# Autodesk Inventor assembly: Сборка1
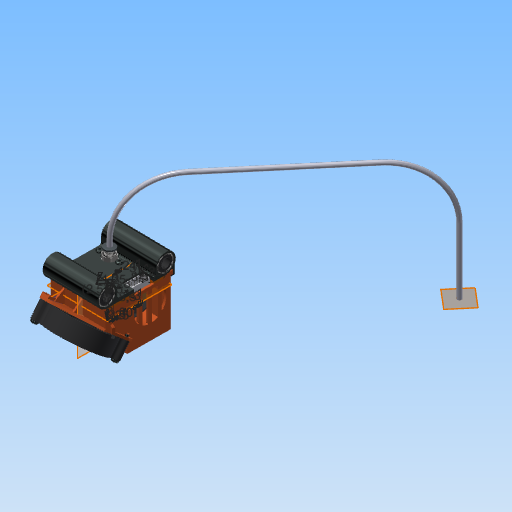
[picture p0: Inventor's stored thumbnail of the model, 512x512]
Saved by Autodesk Inventor 2017 (Build 210142000, 142)
## iProperties
Part Number: Сборка1
Material: Типовые
Document SubType Name: Assembly
Designer: Max
Author: Max
## Documents named in this file (20)
- C:\Users\Max\Desktop\Flying Bear Ghost 5\hotend assembly.iam
- C:\Users\Max\Desktop\Flying Bear Ghost 5\screw m3.ipt
- C:\Users\Max\Desktop\Flying Bear Ghost 5\linear bearing 8x15x24.ipt
- C:\Users\Max\Desktop\Flying Bear Ghost 5\hotend carriage.ipt
- C:\Users\Max\Desktop\Flying Bear Ghost 5\casing 1.ipt
- C:\Users\Max\Desktop\Flying Bear Ghost 5\casing2.ipt
- C:\Users\Max\Desktop\Flying Bear Ghost 5\hotend board.ipt
- C:\Users\Max\Desktop\Flying Bear Ghost 5\radiator Е3DV6.ipt
- C:\Users\Max\Desktop\Flying Bear Ghost 5\thermal barrier.ipt
- C:\Users\Max\Desktop\Flying Bear Ghost 5\fitting 1.ipt
- C:\Users\Max\Desktop\Flying Bear Ghost 5\heating block.ipt
- C:\Users\Max\Desktop\Flying Bear Ghost 5\nozzle 0.4 nozzle.ipt
- C:\Users\Max\Desktop\Flying Bear Ghost 5\thermal sensor.ipt
- C:\Users\Max\Desktop\Flying Bear Ghost 5\thermal sensor1.ipt
- C:\Users\Max\Desktop\Flying Bear Ghost 5\block cover.ipt
- C:\Users\Max\Desktop\Flying Bear Ghost 5\5015 snail blower fan.ipt
- C:\Users\Max\Desktop\Flying Bear Ghost 5\screw m3 long.ipt
- C:\Users\Max\Desktop\Flying Bear Ghost 5\3010-2.ipt
- C:\Users\Max\Desktop\Flying Bear Ghost 5\3010.ipt
- C:\Users\Max\Desktop\Flying Bear Ghost 5\teflon.ipt
## Components (27 placed, 19 different names)
1. hotend carriage:1 — Совмещение:276, Совмещение:277, Совмещение:278, Совмещение:279, Заподлицо:110, Заподлицо:111, Заподлицо:112, Заподлицо:113, Совмещение:282, Совмещение:283, Совмещение:285, Совмещение:287, Совмещение:288, Совмещение:290, Совмещение:291, Совмещение:292, Совмещение:298, Совмещение:299, Совмещение:300, Совмещение:301, Совмещение:317, Совмещение:318, Совмещение:319
2. linear bearing 8x15x24:5 — Совмещение:277, Заподлицо:111
3. linear bearing 8x15x24:6 — Совмещение:278, Заподлицо:110
4. linear bearing 8x15x24:7 — Совмещение:276, Заподлицо:112
5. linear bearing 8x15x24:8 — Совмещение:279, Заподлицо:113
6. casing 1:1 — Совмещение:282, Совмещение:283, Заподлицо:114, Совмещение:284, Совмещение:285, Совмещение:286, Совмещение:289, Совмещение:322
7. casing2:1 — Заподлицо:114, Совмещение:284, Совмещение:286, Угол:7, Совмещение:311, Угол:8, Совмещение:312, Совмещение:313, Совмещение:321, Угол:9
8. hotend board:1 — Совмещение:287, Совмещение:288, Совмещение:289
9. radiator Е3DV6:1 — Совмещение:290, Совмещение:291, Совмещение:292, Совмещение:293, Совмещение:294, Совмещение:297, Совмещение:436
10. thermal barrier:1 — Совмещение:293, Совмещение:294, Совмещение:302, Совмещение:304
11. fitting 1:1 — Совмещение:297, Совмещение:436, Совмещение:437
12. screw m3:45 — Совмещение:298, Совмещение:300
13. screw m3:46 — Совмещение:299, Совмещение:301
14. heating block:1 — Совмещение:302, Совмещение:303, Угол:7, Совмещение:305, Совмещение:306, Заподлицо:116, Совмещение:307, Заподлицо:117, Совмещение:309, Совмещение:310
15. nozzle 0.4 nozzle:1 — Совмещение:303, Совмещение:304, Совмещение:305, Совмещение:308
16. thermal sensor:1 — Совмещение:306, Заподлицо:116
17. thermal sensor1:1 — Совмещение:307, Заподлицо:117
18. block cover:1 — Совмещение:308, Совмещение:309, Совмещение:310
19. 5015 snail blower fan:1 — Совмещение:311, Угол:8, Совмещение:312, Совмещение:313, Совмещение:314, Совмещение:315, Совмещение:316
20. screw m3 long:1 — Совмещение:314, Совмещение:315, Заподлицо:118
21. screw m3 long:2 — Совмещение:316, Заподлицо:118
22. screw m3 long:3 — Совмещение:318, Заподлицо:119
23. screw m3 long:4 — Совмещение:317, Заподлицо:119, Совмещение:319
24. 3010-2:1 — Совмещение:320, Заподлицо:120, Совмещение:322
25. 3010:1 — Совмещение:320, Заподлицо:120, Совмещение:321, Угол:9
26. teflon:1 — Совмещение:437, Совмещение:438, Совмещение:439
27. teflon:2 — Совмещение:438, Совмещение:439
## Relationships (60: Mate 47, Flush 10, Angle 3)
- Совмещение:276 [Mate]: hotend carriage:1 ↔ linear bearing 8x15x24:7
- Совмещение:277 [Mate]: hotend carriage:1 ↔ linear bearing 8x15x24:5
- Совмещение:278 [Mate]: hotend carriage:1 ↔ linear bearing 8x15x24:6
- Совмещение:279 [Mate]: hotend carriage:1 ↔ linear bearing 8x15x24:8
- Заподлицо:110 [Flush]: hotend carriage:1 ↔ linear bearing 8x15x24:6
- Заподлицо:111 [Flush]: hotend carriage:1 ↔ linear bearing 8x15x24:5
- Заподлицо:112 [Flush]: hotend carriage:1 ↔ linear bearing 8x15x24:7
- Заподлицо:113 [Flush]: hotend carriage:1 ↔ linear bearing 8x15x24:8
- Совмещение:282 [Mate]: hotend carriage:1 ↔ casing 1:1
- Совмещение:283 [Mate]: hotend carriage:1 ↔ casing 1:1
- Заподлицо:114 [Flush]: casing 1:1 ↔ casing2:1
- Совмещение:284 [Mate]: casing 1:1 ↔ casing2:1
- Совмещение:285 [Mate]: hotend carriage:1 ↔ casing 1:1
- Совмещение:286 [Mate]: casing 1:1 ↔ casing2:1
- Совмещение:287 [Mate]: hotend carriage:1 ↔ hotend board:1
- Совмещение:288 [Mate]: hotend carriage:1 ↔ hotend board:1
- Совмещение:289 [Mate]: casing 1:1 ↔ hotend board:1
- Совмещение:290 [Mate]: hotend carriage:1 ↔ radiator Е3DV6:1
- Совмещение:291 [Mate]: hotend carriage:1 ↔ radiator Е3DV6:1
- Совмещение:292 [Mate]: hotend carriage:1 ↔ radiator Е3DV6:1
- Совмещение:293 [Mate]: radiator Е3DV6:1 ↔ thermal barrier:1
- Совмещение:294 [Mate]: radiator Е3DV6:1 ↔ thermal barrier:1
- Совмещение:297 [Mate]: radiator Е3DV6:1 ↔ fitting 1:1
- Совмещение:298 [Mate]: hotend carriage:1 ↔ screw m3:45
- Совмещение:299 [Mate]: hotend carriage:1 ↔ screw m3:46
- Совмещение:300 [Mate]: hotend carriage:1 ↔ screw m3:45
- Совмещение:301 [Mate]: hotend carriage:1 ↔ screw m3:46
- Совмещение:302 [Mate]: thermal barrier:1 ↔ heating block:1
- Совмещение:303 [Mate]: heating block:1 ↔ nozzle 0.4 nozzle:1
- Совмещение:304 [Mate]: thermal barrier:1 ↔ nozzle 0.4 nozzle:1
- Угол:7 [Angle] (0 deg): casing2:1 ↔ heating block:1
- Совмещение:305 [Mate] (0.5 mm): heating block:1 ↔ nozzle 0.4 nozzle:1
- Совмещение:306 [Mate]: heating block:1 ↔ thermal sensor:1
- Заподлицо:116 [Flush] (-1 mm): heating block:1 ↔ thermal sensor:1
- Совмещение:307 [Mate]: heating block:1 ↔ thermal sensor1:1
- Заподлицо:117 [Flush]: heating block:1 ↔ thermal sensor1:1
- Совмещение:308 [Mate]: nozzle 0.4 nozzle:1 ↔ block cover:1
- Совмещение:309 [Mate]: heating block:1 ↔ block cover:1
- Совмещение:310 [Mate]: heating block:1 ↔ block cover:1
- Совмещение:311 [Mate]: casing2:1 ↔ 5015 snail blower fan:1
- Угол:8 [Angle] (0 deg): casing2:1 ↔ 5015 snail blower fan:1
- Совмещение:312 [Mate]: casing2:1 ↔ 5015 snail blower fan:1
- Совмещение:313 [Mate]: casing2:1 ↔ 5015 snail blower fan:1
- Совмещение:314 [Mate]: 5015 snail blower fan:1 ↔ screw m3 long:1
- Совмещение:315 [Mate]: 5015 snail blower fan:1 ↔ screw m3 long:1
- Совмещение:316 [Mate]: 5015 snail blower fan:1 ↔ screw m3 long:2
- Заподлицо:118 [Flush]: screw m3 long:1 ↔ screw m3 long:2
- Совмещение:317 [Mate]: hotend carriage:1 ↔ screw m3 long:4
- Совмещение:318 [Mate]: hotend carriage:1 ↔ screw m3 long:3
- Заподлицо:119 [Flush]: screw m3 long:3 ↔ screw m3 long:4
- Совмещение:319 [Mate]: hotend carriage:1 ↔ screw m3 long:4
- Совмещение:320 [Mate]: 3010-2:1 ↔ 3010:1
- Заподлицо:120 [Flush]: 3010-2:1 ↔ 3010:1
- Совмещение:321 [Mate]: casing2:1 ↔ 3010:1
- Угол:9 [Angle] (0 deg): casing2:1 ↔ 3010:1
- Совмещение:322 [Mate]: casing 1:1 ↔ 3010-2:1
- Совмещение:436 [Mate]: radiator Е3DV6:1 ↔ fitting 1:1
- Совмещение:437 [Mate]: fitting 1:1 ↔ teflon:1
- Совмещение:438 [Mate]: teflon:1 ↔ teflon:2
- Совмещение:439 [Mate]: teflon:1 ↔ teflon:2
